# Autodesk Inventor assembly: Baugruppe
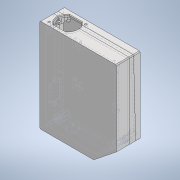
[picture p0: Inventor's stored thumbnail of the model, 180x180]
Saved by Autodesk Inventor 2020 (Build 240168000, 168)
## iProperties
Created: 2020-04-10
Part Number: Baugruppe
Document SubType Name: Assembly
Designer: Windooof
Author: Windooof
## Documents named in this file (3)
- C:\Users\Windooof\Documents\Inventor\Facharbeit\Assembly.iam
- C:\Users\Windooof\Documents\Inventor\Facharbeit\Case.ipt
- C:\Users\Windooof\Documents\Inventor\Facharbeit\CaseLidShape.ipt
## Components (2 placed, 2 different names)
1. Case:1 — Fluchtend:1, Fluchtend:2, Passend:1
2. CaseLidShape:1 — Fluchtend:1, Fluchtend:2, Passend:1
## Relationships (3: Flush 2, Mate 1)
- Fluchtend:1 [Flush]: Case:1 ↔ CaseLidShape:1
- Fluchtend:2 [Flush]: Case:1 ↔ CaseLidShape:1
- Passend:1 [Mate]: Case:1 ↔ CaseLidShape:1
